# Autodesk Inventor assembly: Base
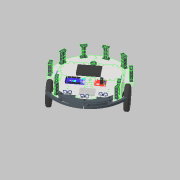
[picture p0: Inventor's stored thumbnail of the model, 180x180]
Saved by Autodesk Inventor 2017 (Build 210142000, 142)
## iProperties
Created: 2017-03-11
Part Number: Base
Document SubType Name: Assembly
Designer: zallen
Author: zallen
## Documents named in this file (10)
- C:\Users\zallen\Documents\GitHub\cr-laundry-robot\src\Base\Base.iam
- C:\Users\zallen\Documents\GitHub\cr-laundry-robot\src\Base\Swivel Wheel.ipt
- C:\Users\zallen\Documents\GitHub\cr-laundry-robot\lib\HC-SR04 Ultasonic Sensor\Sensor Ultrasónico.ipt
- C:\Users\zallen\Documents\GitHub\cr-laundry-robot\lib\Breadboard\breadboard_350_pos_asm.iam
- C:\Users\zallen\Documents\GitHub\cr-laundry-robot\lib\Arduino Mega 2560\Arduino Mega 2560.ipt
- C:\Users\zallen\Documents\GitHub\cr-laundry-robot\lib\L298n\Драйвер двигателей L298N.ipt
- C:\Users\zallen\Documents\GitHub\cr-laundry-robot\src\Base\Drive Wheel Assembly\DriveAssembly.iam
- C:\Users\zallen\Documents\GitHub\cr-laundry-robot\src\Base\Battery Pack Assembly\BatteryPackAssembly.iam
- C:\Users\zallen\Documents\GitHub\cr-laundry-robot\src\Base\Bumper Assembly\Bumper Assembly.iam
- C:\Users\zallen\Documents\GitHub\cr-laundry-robot\src\Base\Chassis - Modular\Chassis.iam
## Components (13 placed, 9 different names)
1. Swivel Wheel:1 — Mate:75, Mate:76
2. Sensor Ultrasónico:1 — Mate:77, Mate:78, Mate:79
3. Sensor Ultrasónico:2 — Mate:80, Mate:81
4. Sensor Ultrasónico:3 — Mate:82, Mate:83
5. Sensor Ultrasónico:4 — Mate:84, Mate:85
6. Sensor Ultrasónico:5 — Mate:86, Mate:87, Mate:88
7. breadboard_350_pos_asm:1 [sub-assembly] — Mate:89, Mate:92, Mate:94
8. Arduino Mega 2560:1 — Mate:90, Mate:91, Mate:98
9. L298N:1 — Mate:95, Mate:96, Mate:97
10. DriveAssembly:1 [sub-assembly] — Mate:72, Mate:74
11. BatteryPackAssembly:1 [sub-assembly] — Mate:99, Mate:100
12. Bumper Assembly:1 [sub-assembly] — Mate:67, Mate:101, Mate:102
13. Chassis:1 [sub-assembly] — Mate:66, Mate:67, Mate:72, Mate:74, Mate:75, Mate:76, Mate:77, Mate:78, Mate:79, Mate:80, Mate:81, Mate:82, Mate:83, Mate:84, Mate:85, Mate:86, Mate:87, Mate:88, Mate:89, Mate:90, Mate:91, Mate:92, Mate:94, Mate:95, Mate:96, Mate:97, Mate:98, Mate:99, Mate:100, Mate:101, Mate:102
## Relationships (31: Mate 31)
- Mate:66: Chassis:1
- Mate:67: Bumper Assembly:1 ↔ Chassis:1
- Mate:72: DriveAssembly:1 ↔ Chassis:1
- Mate:74: DriveAssembly:1 ↔ Chassis:1
- Mate:75: Swivel Wheel:1 ↔ Chassis:1
- Mate:76: Swivel Wheel:1 ↔ Chassis:1
- Mate:77: Sensor Ultrasónico:1 ↔ Chassis:1
- Mate:78: Sensor Ultrasónico:1 ↔ Chassis:1
- Mate:79: Sensor Ultrasónico:1 ↔ Chassis:1
- Mate:80: Sensor Ultrasónico:2 ↔ Chassis:1
- Mate:81: Sensor Ultrasónico:2 ↔ Chassis:1
- Mate:82: Sensor Ultrasónico:3 ↔ Chassis:1
- Mate:83: Sensor Ultrasónico:3 ↔ Chassis:1
- Mate:84: Sensor Ultrasónico:4 ↔ Chassis:1
- Mate:85: Sensor Ultrasónico:4 ↔ Chassis:1
- Mate:86: Sensor Ultrasónico:5 ↔ Chassis:1
- Mate:87: Sensor Ultrasónico:5 ↔ Chassis:1
- Mate:88: Sensor Ultrasónico:5 ↔ Chassis:1
- Mate:89: breadboard_350_pos_asm:1 ↔ Chassis:1
- Mate:90: Arduino Mega 2560:1 ↔ Chassis:1
- Mate:91: Arduino Mega 2560:1 ↔ Chassis:1
- Mate:92: breadboard_350_pos_asm:1 ↔ Chassis:1
- Mate:94: breadboard_350_pos_asm:1 ↔ Chassis:1
- Mate:95: L298N:1 ↔ Chassis:1
- Mate:96: L298N:1 ↔ Chassis:1
- Mate:97: L298N:1 ↔ Chassis:1
- Mate:98: Arduino Mega 2560:1 ↔ Chassis:1
- Mate:99: BatteryPackAssembly:1 ↔ Chassis:1
- Mate:100: BatteryPackAssembly:1 ↔ Chassis:1
- Mate:101: Bumper Assembly:1 ↔ Chassis:1
- Mate:102: Bumper Assembly:1 ↔ Chassis:1
